# Autodesk Inventor assembly: 总装01
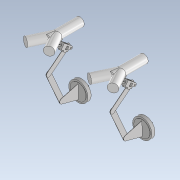
[picture p0: Inventor's stored thumbnail of the model, 180x180]
Saved by Autodesk Inventor 2022.5 (Build 265521000, 521)
## iProperties
Created: 2024-11-13
Part Number: 总装01
Document SubType Name: Assembly
Designer: Gagouking
Author: Gagouking
## Documents named in this file (2)
- D:\Documents\好玩的\水下机器人\总装01.iam
- D:\Documents\好玩的\水下机器人\机械臂.iam
## Components (2 placed, 1 different names)
1. 机械臂:1 [sub-assembly] — 表面齐平:1, 表面齐平:2, 配合:1
2. 机械臂:2 [sub-assembly] — 表面齐平:1, 表面齐平:2, 配合:1
## Relationships (3: Flush 2, Mate 1)
- 表面齐平:1 [Flush]: 机械臂:1 ↔ 机械臂:2
- 表面齐平:2 [Flush]: 机械臂:1 ↔ 机械臂:2
- 配合:1 [Mate] (200 mm): 机械臂:1 ↔ 机械臂:2
